# Autodesk Inventor assembly: Tape Winch
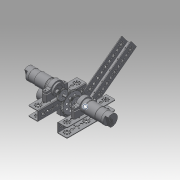
[picture p0: Inventor's stored thumbnail of the model, 180x180]
Saved by Autodesk Inventor 2016 (Build 200138000, 138)
## iProperties
Created: 2016-02-10
Part Number: Tape Winch
Document SubType Name: Assembly
Designer: Delta
Author: Delta
## Documents named in this file (7)
- C:\Robotics\CAD\2015-16\custom cad parts\Tape Winch.iam
- C:\Robotics\CAD\2015-16\COTSParts\Tetrix\Tetrix channel 160mm.ipt
- C:\Robotics\CAD\2015-16\COTSParts\Tetrix\Tetrix Gear 80T.ipt
- C:\Robotics\CAD\2015-16\COTSParts\Tetrix\Tetrix Hub - axle.ipt
- C:\Robotics\CAD\2015-16\COTSParts\Tetrix\Tetrix motor mount.ipt
- C:\Robotics\CAD\2015-16\COTSParts\Motors\Andymark 2964  NeveRest 40 Motor.ipt
- C:\Robotics\CAD\2015-16\COTSParts\Tetrix\Tetrix Gear 40T.ipt
## Components (14 placed, 6 different names)
1. Tetrix channel 160mm:1 — Mate:2, Mate:3
2. Tetrix channel 160mm:2 — Mate:1, Flush:1, Flush:2, Mate:2, Mate:3, Mate:4, Mate:6, Mate:13, Mate:14, Mate:15, Mate:21, Mate:22, Mate:23
3. Tetrix channel 160mm:3 — Mate:1, Flush:1, Flush:2, Mate:5, Mate:7, Mate:10, Mate:11, Mate:12
4. Tetrix Gear 80T:1 — Mate:5, Mate:7, Flush:6
5. Tetrix Gear 80T:2 — Mate:4, Mate:6, Mate:8, Mate:9, Flush:5
6. Tetrix Hub - axle:1 — Mate:8, Mate:9
7. Tetrix motor mount:1 — Mate:10, Mate:11, Mate:12, Mate:16, Flush:3
8. Tetrix motor mount:2 — Mate:13, Mate:14, Mate:15, Mate:18, Flush:4
9. Andymark 2964  NeveRest 40 Motor:1 — Mate:16, Flush:3, Mate:17, Mate:20
10. Andymark 2964  NeveRest 40 Motor:2 — Mate:17, Mate:18, Flush:4, Mate:19
11. Tetrix Gear 40T:1 — Mate:20, Flush:6
12. Tetrix Gear 40T:2 — Mate:19, Flush:5
13. Tetrix motor mount:3 — Mate:21, Mate:22, Mate:23, Mate:25, Flush:7
14. Andymark 2964  NeveRest 40 Motor:3 — Mate:25, Flush:7
## Relationships (31: Mate 24, Flush 7)
- Mate:1 (63.5 mm): Tetrix channel 160mm:2 ↔ Tetrix channel 160mm:3
- Flush:1: Tetrix channel 160mm:2 ↔ Tetrix channel 160mm:3
- Flush:2: Tetrix channel 160mm:2 ↔ Tetrix channel 160mm:3
- Mate:2 (19.558 mm): Tetrix channel 160mm:1 ↔ Tetrix channel 160mm:2
- Mate:3: Tetrix channel 160mm:1 ↔ Tetrix channel 160mm:2
- Mate:4 (12 mm): Tetrix channel 160mm:2 ↔ Tetrix Gear 80T:2
- Mate:5 (4 mm): Tetrix channel 160mm:3 ↔ Tetrix Gear 80T:1
- Mate:6: Tetrix channel 160mm:2 ↔ Tetrix Gear 80T:2
- Mate:7: Tetrix channel 160mm:3 ↔ Tetrix Gear 80T:1
- Mate:8: Tetrix Gear 80T:2 ↔ Tetrix Hub - axle:1
- Mate:9: Tetrix Gear 80T:2 ↔ Tetrix Hub - axle:1
- Mate:10: Tetrix channel 160mm:3 ↔ Tetrix motor mount:1
- Mate:11: Tetrix channel 160mm:3 ↔ Tetrix motor mount:1
- Mate:12: Tetrix channel 160mm:3 ↔ Tetrix motor mount:1
- Mate:13: Tetrix channel 160mm:2 ↔ Tetrix motor mount:2
- Mate:14: Tetrix channel 160mm:2 ↔ Tetrix motor mount:2
- Mate:15: Tetrix channel 160mm:2 ↔ Tetrix motor mount:2
- Mate:16: Tetrix motor mount:1 ↔ Andymark 2964  NeveRest 40 Motor:1
- Flush:3 (-2 mm): Tetrix motor mount:1 ↔ Andymark 2964  NeveRest 40 Motor:1
- Mate:17: Andymark 2964  NeveRest 40 Motor:1 ↔ Andymark 2964  NeveRest 40 Motor:2
- Mate:18: Tetrix motor mount:2 ↔ Andymark 2964  NeveRest 40 Motor:2
- Flush:4 (6 mm): Tetrix motor mount:2 ↔ Andymark 2964  NeveRest 40 Motor:2
- Mate:19: Andymark 2964  NeveRest 40 Motor:2 ↔ Tetrix Gear 40T:2
- Mate:20: Andymark 2964  NeveRest 40 Motor:1 ↔ Tetrix Gear 40T:1
- Flush:5: Tetrix Gear 80T:2 ↔ Tetrix Gear 40T:2
- Flush:6: Tetrix Gear 80T:1 ↔ Tetrix Gear 40T:1
- Mate:21: Tetrix channel 160mm:2 ↔ Tetrix motor mount:3
- Mate:22: Tetrix channel 160mm:2 ↔ Tetrix motor mount:3
- Mate:23: Tetrix channel 160mm:2 ↔ Tetrix motor mount:3
- Mate:25: Tetrix motor mount:3 ↔ Andymark 2964  NeveRest 40 Motor:3
- Flush:7 (3 mm): Tetrix motor mount:3 ↔ Andymark 2964  NeveRest 40 Motor:3
